# Autodesk Inventor assembly: zlozenie
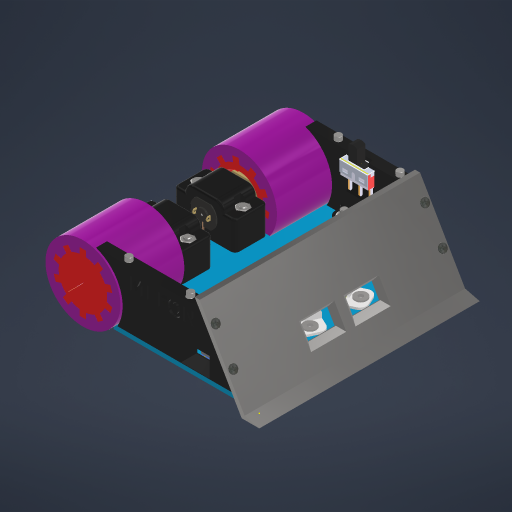
[picture p0: Inventor's stored thumbnail of the model, 512x512]
Saved by Autodesk Inventor 2024 (Build 280153000, 153)
## iProperties
Created: 2024-05-23
Part Number: zlozenie
Document SubType Name: Assembly
Designer: Adam
Mass: 276.182 g
Surface Area: 1098.73 cm^2
Volume: 114.459 cm^3
Density: 2.41293 g/cm^3
Author: Adam
## Documents named in this file (28)
- C:\Users\pryst\Desktop\KoNaR\Warsztaty\minisumo\model\zlozenie.iam
- C:\Users\pryst\Desktop\KoNaR\Warsztaty\minisumo\model\modele_stp\modele_stp\N20 DC MOTOR\N20 DC MOTOR.ipt
- C:\Users\pryst\Desktop\KoNaR\Warsztaty\minisumo\model\modele_stp\modele_stp\TOF VL53L0X\TOF VL53L0X.ipt
- C:\Users\pryst\Desktop\KoNaR\Warsztaty\minisumo\model\felga.ipt
- C:\Users\pryst\Desktop\KoNaR\Warsztaty\minisumo\model\podstawa.ipt
- C:\Users\pryst\Desktop\KoNaR\Warsztaty\minisumo\model\mocowanie_silnika.ipt
- C:\Users\pryst\Desktop\KoNaR\Warsztaty\minisumo\model\podstawka silnika.ipt
- C:\Users\pryst\Desktop\KoNaR\Warsztaty\minisumo\model\opona.ipt
- C:\Users\pryst\Desktop\KoNaR\Warsztaty\minisumo\model\lemiesz.ipt
- C:\Users\pryst\Desktop\KoNaR\Warsztaty\minisumo\model\modele_stp\modele_stp\N20 DC MOTOR\N20 DC MOTOR_CPY.ipt
- C:\Users\pryst\Desktop\KoNaR\Warsztaty\minisumo\model\mocowanie_silnika_CPY.ipt
- C:\Users\pryst\Desktop\KoNaR\Warsztaty\minisumo\model\podstawka silnika_CPY.ipt
- C:\Users\pryst\Desktop\KoNaR\Warsztaty\minisumo\model\mocowanie_tofa.ipt
- C:\Users\pryst\Desktop\KoNaR\Warsztaty\minisumo\model\modele_stp\modele_stp\TOF VL53L0X\TOF VL53L0X_CPY.ipt
- C:\Users\pryst\Desktop\KoNaR\Warsztaty\minisumo\model\modele_stp\modele_stp\TOF VL53L0X\TOF VL53L0X_CPY1.ipt
- C:\Users\pryst\Desktop\KoNaR\Warsztaty\minisumo\model\modele_stp\modele_stp\TOF VL53L0X\TOF VL53L0X_CPY_CPY.ipt
- C:\Users\pryst\Desktop\KoNaR\Warsztaty\minisumo\model\bok_lewy.ipt
- C:\Users\pryst\Desktop\KoNaR\Warsztaty\minisumo\model\bok_prawy.ipt
- C:\Users\pryst\Desktop\KoNaR\Warsztaty\minisumo\model\podkladka.ipt
- C:\Users\pryst\Documents\Inventor\Content Center Files\R2024\en-US\DIN 934\DIN 934 - M3 x 0,5.ipt
- C:\Users\pryst\Documents\Inventor\Content Center Files\R2024\en-US\DIN 7991(1)\DIN 7991 - M3  x  8.ipt
- C:\Users\pryst\Documents\Inventor\Content Center Files\R2024\en-US\ANSI B18.3.4M(2)\ANSI B18.3.4M - M3 x 0.5 x 10(1).ipt
- C:\Users\pryst\Documents\Inventor\Content Center Files\R2024\en-US\DIN 7991(1)\DIN 7991 - M3  x  16.ipt
- C:\Users\pryst\Documents\Inventor\Content Center Files\R2024\en-US\ISO 7050 - C-Z(1)\DIN EN ISO 7050 - ST2,2 x 4,5 - C - Z.ipt
- C:\Users\pryst\Desktop\KoNaR\Warsztaty\minisumo\model\porywa.ipt
- C:\Users\pryst\Desktop\KoNaR\Warsztaty\minisumo\model\wlacznik.ipt
- C:\Users\pryst\Desktop\KoNaR\Warsztaty\minisumo\model\magnes.ipt
- C:\Users\pryst\Desktop\KoNaR\Warsztaty\minisumo\model\mocowanie_tofa - Copy.ipt
## Components (61 placed, 27 different names)
1. N20 DC MOTOR:1 — Insert:1, Mate:5, Mate:6
2. TOF VL53L0X:1 — Mate:20, Insert:12
3. felga:1 — Insert:1, Insert:3
4. podstawa:1 — Flush:2, Mate:9, Mate:13, Flush:9, Mate:14, Flush:12, Mate:18, Mate:20, Angle:1, Flush:14, Mate:22, Mate:25, Flush:18, Flush:19, Flush:20, Mate:26, Flush:21, Flush:22, Mate:27, Insert:20, Insert:21, Insert:32, Insert:33, Insert:34, Mate:32, Mate:33, Mate:40, Mate:41, Mate:42, Mate:43, Insert:44, Insert:45, Insert:48, Insert:50
5. mocowanie_silnika:1 — Mate:8, Flush:4, Flush:5, Insert:22, Insert:23
6. podstawka silnika:1 — Flush:2, Mate:5, Mate:6, Mate:8, Flush:4, Mate:9, Flush:5, Mate:14, Flush:13
7. opona:1 — Insert:3
8. lemiesz:1 — Mate:13, Flush:9, Flush:14, Mate:48, Mate:49, Mate:50, Mate:51, Mate:53
9. N20 DC MOTOR_CPY:1 — Mate:16, Mate:17, Mate:19, Insert:11
10. mocowanie_silnika_CPY:1 — Flush:10, Flush:11, Mate:15, Insert:24, Insert:25
11. podstawka silnika_CPY:1 — Flush:10, Flush:11, Mate:15, Mate:16, Mate:17, Flush:12, Mate:18, Flush:13, Mate:19
12. mocowanie_tofa:1 — Angle:1, Insert:12, Insert:21, Mate:45
13. TOF VL53L0X_CPY:1 — Mate:69, Insert:47
14. TOF VL53L0X_CPY1:1 — Insert:13
15. TOF VL53L0X_CPY_CPY:1 — Mate:70, Insert:49
16. felga:2 — Insert:10, Insert:11, Mate:68
17. opona:2 — Insert:10, Mate:68
18. mocowanie_tofa:2 — Mate:22, Insert:13, Insert:20, Mate:46
19. bok_lewy:1 — Mate:25, Flush:18, Flush:19, Insert:27, Mate:58, Mate:59, Mate:60, Mate:61, Insert:40, Insert:41
20. bok_prawy:1 — Flush:20, Mate:26, Flush:21, Insert:26, Flush:23, Insert:42, Insert:43
21. podkladka:1 — Mate:27
22. podkladka:2
23. podkladka:3
24. DIN 934 - replaced by DIN EN 24032/28673/28674 M3:1 — Insert:22
25. DIN 934 - replaced by DIN EN 24032/28673/28674 M3:2 — Insert:23
26. DIN 934 - replaced by DIN EN 24032/28673/28674 M3:3 — Insert:24
27. DIN 934 - replaced by DIN EN 24032/28673/28674 M3:4 — Insert:25
28. DIN 934 - replaced by DIN EN 24032/28673/28674 M3:5 — Insert:26
29. DIN 934 - replaced by DIN EN 24032/28673/28674 M3:6 — Insert:27
30. DIN 934 - replaced by DIN EN 24032/28673/28674 M3:11 — Insert:32
31. DIN 934 - replaced by DIN EN 24032/28673/28674 M3:12 — Insert:33
32. DIN 934 - replaced by DIN EN 24032/28673/28674 M3:13 — Insert:34
33. DIN 7991 - replaced by DIN EN ISO 10642 M3  x  8:2 — Mate:32
34. DIN 7991 - replaced by DIN EN ISO 10642 M3  x  8:3 — Mate:33
35. DIN 7991 - replaced by DIN EN ISO 10642 M3  x  16:1 — Mate:40
36. DIN 7991 - replaced by DIN EN ISO 10642 M3  x  16:2 — Mate:41
37. DIN 7991 - replaced by DIN EN ISO 10642 M3  x  16:3 — Mate:43
38. DIN 7991 - replaced by DIN EN ISO 10642 M3  x  16:4 — Mate:42
39. DIN 7991 - replaced by DIN EN ISO 10642 M3  x  8:5 — Mate:45
40. DIN 7991 - replaced by DIN EN ISO 10642 M3  x  8:6 — Mate:46
41. DIN EN ISO 7050 - C-Z ST2,2 x 4,5 - C - Z:1 — Mate:48
42. DIN EN ISO 7050 - C-Z ST2,2 x 4,5 - C - Z:2 — Mate:49
43. DIN EN ISO 7050 - C-Z ST2,2 x 4,5 - C - Z:3 — Mate:50
44. DIN EN ISO 7050 - C-Z ST2,2 x 4,5 - C - Z:4 — Mate:51
45. porywa:1 — Flush:23, Mate:53, Mate:61, Insert:36, Insert:37, Insert:38, Insert:39
46. wlacznik:1 — Mate:58, Mate:59, Mate:60
47. magnes:1 — Insert:38
48. magnes:2 — Insert:39
49. magnes:3 — Insert:37
50. magnes:4 — Insert:36
51. magnes:5 — Insert:40
52. magnes:6 — Insert:41
53. magnes:7 — Insert:42
54. magnes:8 — Insert:43
55. DIN 934 - replaced by DIN EN 24032/28673/28674 M3:15 — Insert:44
56. DIN 934 - replaced by DIN EN 24032/28673/28674 M3:16 — Insert:45
57. Forged Hexagon Socket Button Head Cap Screw - Metric M3 x 0.5 x 10:2
58. Forged Hexagon Socket Button Head Cap Screw - Metric M3 x 0.5 x 10:3
59. Forged Hexagon Socket Button Head Cap Screw - Metric M3 x 0.5 x 10:4
60. mocowanie_tofa - Copy:1 — Mate:69, Insert:47, Insert:48
61. mocowanie_tofa - Copy:2 — Mate:70, Insert:49, Insert:50
## Relationships (83: Mate 36, Insert 31, Flush 15, Angle 1)
- Insert:1: N20 DC MOTOR:1 ↔ felga:1
- Flush:2: podstawa:1 ↔ podstawka silnika:1
- Mate:5: N20 DC MOTOR:1 ↔ podstawka silnika:1
- Mate:6: N20 DC MOTOR:1 ↔ podstawka silnika:1
- Mate:8: mocowanie_silnika:1 ↔ podstawka silnika:1
- Flush:4: mocowanie_silnika:1 ↔ podstawka silnika:1
- Mate:9: podstawa:1 ↔ podstawka silnika:1
- Flush:5: mocowanie_silnika:1 ↔ podstawka silnika:1
- Insert:3: felga:1 ↔ opona:1
- Mate:13: podstawa:1 ↔ lemiesz:1
- Flush:9: podstawa:1 ↔ lemiesz:1
- Mate:14: podstawa:1 ↔ podstawka silnika:1
- Flush:10: mocowanie_silnika_CPY:1 ↔ podstawka silnika_CPY:1
- Flush:11: mocowanie_silnika_CPY:1 ↔ podstawka silnika_CPY:1
- Mate:15: mocowanie_silnika_CPY:1 ↔ podstawka silnika_CPY:1
- Mate:16: N20 DC MOTOR_CPY:1 ↔ podstawka silnika_CPY:1
- Mate:17: N20 DC MOTOR_CPY:1 ↔ podstawka silnika_CPY:1
- Flush:12: podstawa:1 ↔ podstawka silnika_CPY:1
- Mate:18: podstawa:1 ↔ podstawka silnika_CPY:1
- Flush:13: podstawka silnika:1 ↔ podstawka silnika_CPY:1
- Mate:19: N20 DC MOTOR_CPY:1 ↔ podstawka silnika_CPY:1
- Mate:20: TOF VL53L0X:1 ↔ podstawa:1
- Angle:1 (25 deg): podstawa:1 ↔ mocowanie_tofa:1
- Flush:14 (6 mm): podstawa:1 ↔ lemiesz:1
- Insert:10: felga:2 ↔ opona:2
- Insert:11: N20 DC MOTOR_CPY:1 ↔ felga:2
- Insert:12: TOF VL53L0X:1 ↔ mocowanie_tofa:1
- Mate:22: podstawa:1 ↔ mocowanie_tofa:2
- Insert:13: TOF VL53L0X_CPY1:1 ↔ mocowanie_tofa:2
- Mate:25: podstawa:1 ↔ bok_lewy:1
- Flush:18: podstawa:1 ↔ bok_lewy:1
- Flush:19: podstawa:1 ↔ bok_lewy:1
- Flush:20: podstawa:1 ↔ bok_prawy:1
- Mate:26: podstawa:1 ↔ bok_prawy:1
- Flush:21: podstawa:1 ↔ bok_prawy:1
- Flush:22 (15 mm): podstawa:1
- Mate:27: podstawa:1 ↔ podkladka:1
- Insert:20: podstawa:1 ↔ mocowanie_tofa:2
- Insert:21: podstawa:1 ↔ mocowanie_tofa:1
- Insert:22: mocowanie_silnika:1 ↔ DIN 934 - replaced by DIN EN 24032/28673/28674 M3:1
- Insert:23: mocowanie_silnika:1 ↔ DIN 934 - replaced by DIN EN 24032/28673/28674 M3:2
- Insert:24: mocowanie_silnika_CPY:1 ↔ DIN 934 - replaced by DIN EN 24032/28673/28674 M3:3
- Insert:25: mocowanie_silnika_CPY:1 ↔ DIN 934 - replaced by DIN EN 24032/28673/28674 M3:4
- Insert:26: bok_prawy:1 ↔ DIN 934 - replaced by DIN EN 24032/28673/28674 M3:5
- Insert:27: bok_lewy:1 ↔ DIN 934 - replaced by DIN EN 24032/28673/28674 M3:6
- Insert:32: podstawa:1 ↔ DIN 934 - replaced by DIN EN 24032/28673/28674 M3:11
- Insert:33: podstawa:1 ↔ DIN 934 - replaced by DIN EN 24032/28673/28674 M3:12
- Insert:34: podstawa:1 ↔ DIN 934 - replaced by DIN EN 24032/28673/28674 M3:13
- Mate:32: podstawa:1 ↔ DIN 7991 - replaced by DIN EN ISO 10642 M3  x  8:2
- Mate:33: podstawa:1 ↔ DIN 7991 - replaced by DIN EN ISO 10642 M3  x  8:3
- Mate:40: podstawa:1 ↔ DIN 7991 - replaced by DIN EN ISO 10642 M3  x  16:1
- Mate:41: podstawa:1 ↔ DIN 7991 - replaced by DIN EN ISO 10642 M3  x  16:2
- Mate:42: podstawa:1 ↔ DIN 7991 - replaced by DIN EN ISO 10642 M3  x  16:4
- Mate:43: podstawa:1 ↔ DIN 7991 - replaced by DIN EN ISO 10642 M3  x  16:3
- Mate:45: mocowanie_tofa:1 ↔ DIN 7991 - replaced by DIN EN ISO 10642 M3  x  8:5
- Mate:46: mocowanie_tofa:2 ↔ DIN 7991 - replaced by DIN EN ISO 10642 M3  x  8:6
- Mate:48: lemiesz:1 ↔ DIN EN ISO 7050 - C-Z ST2,2 x 4,5 - C - Z:1
- Mate:49: lemiesz:1 ↔ DIN EN ISO 7050 - C-Z ST2,2 x 4,5 - C - Z:2
- Mate:50: lemiesz:1 ↔ DIN EN ISO 7050 - C-Z ST2,2 x 4,5 - C - Z:3
- Mate:51: lemiesz:1 ↔ DIN EN ISO 7050 - C-Z ST2,2 x 4,5 - C - Z:4
- Flush:23: bok_prawy:1 ↔ porywa:1
- Mate:53: lemiesz:1 ↔ porywa:1
- Mate:58: bok_lewy:1 ↔ wlacznik:1
- Mate:59: bok_lewy:1 ↔ wlacznik:1
- Mate:60: bok_lewy:1 ↔ wlacznik:1
- Mate:61: bok_lewy:1 ↔ porywa:1
- Insert:36: porywa:1 ↔ magnes:4
- Insert:37: porywa:1 ↔ magnes:3
- Insert:38: porywa:1 ↔ magnes:1
- Insert:39: porywa:1 ↔ magnes:2
- Insert:40: bok_lewy:1 ↔ magnes:5
- Insert:41: bok_lewy:1 ↔ magnes:6
- Insert:42: bok_prawy:1 ↔ magnes:7
- Insert:43: bok_prawy:1 ↔ magnes:8
- Insert:44: podstawa:1 ↔ DIN 934 - replaced by DIN EN 24032/28673/28674 M3:15
- Insert:45: podstawa:1 ↔ DIN 934 - replaced by DIN EN 24032/28673/28674 M3:16
- Mate:68: felga:2 ↔ opona:2
- Mate:69: TOF VL53L0X_CPY:1 ↔ mocowanie_tofa - Copy:1
- Insert:47: TOF VL53L0X_CPY:1 ↔ mocowanie_tofa - Copy:1
- Insert:48: podstawa:1 ↔ mocowanie_tofa - Copy:1
- Mate:70: TOF VL53L0X_CPY_CPY:1 ↔ mocowanie_tofa - Copy:2
- Insert:49: TOF VL53L0X_CPY_CPY:1 ↔ mocowanie_tofa - Copy:2
- Insert:50: podstawa:1 ↔ mocowanie_tofa - Copy:2
